# Autodesk Inventor assembly: robot
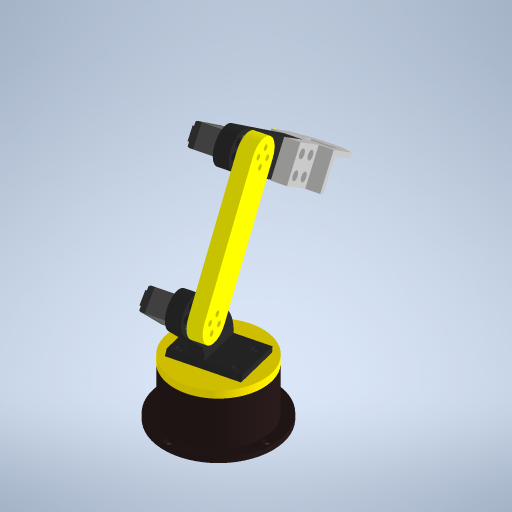
[picture p0: Inventor's stored thumbnail of the model, 512x512]
Saved by Autodesk Inventor 2024.2 (Build 282272000, 272)
## iProperties
Created: 2023-11-10
Part Number: robot
Document SubType Name: Assembly
Designer: nosal
Author: nosal
## Documents named in this file (8)
- C:\Users\nosal\OneDrive\Pulpit\projekty 3d\Inżynierka\Robot2\robot.iam
- C:\Users\nosal\OneDrive\Pulpit\projekty 3d\Inżynierka\Robot2\Podstawa1.ipt
- C:\Users\nosal\OneDrive\Pulpit\projekty 3d\Inżynierka\Robot2\silnik\MG_996R.iam
- C:\Users\nosal\OneDrive\Pulpit\projekty 3d\Inżynierka\Robot2\Podstawa2.ipt
- C:\Users\nosal\OneDrive\Pulpit\projekty 3d\Inżynierka\Robot2\Ramie1.ipt
- C:\Users\nosal\OneDrive\Pulpit\projekty 3d\Inżynierka\Robot2\Ramie2.ipt
- C:\Users\nosal\OneDrive\Pulpit\projekty 3d\Inżynierka\Robot2\Ramie3.ipt
- C:\Users\nosal\OneDrive\Pulpit\projekty 3d\Inżynierka\Robot2\chwytak\podstawachwytak.ipt
## Components (9 placed, 7 different names)
1. Podstawa1:1 — Sztywne:1
2. MG_996R:1 [sub-assembly] — Sztywne:1, Obrotowe:1
3. Podstawa2:1 — Obrotowe:1, Sztywne:2
4. Ramie1:1 — Sztywne:2, Obrotowe:2, Sztywne:3
5. MG_996R:2 [sub-assembly] — Obrotowe:2, Sztywne:3, Obrotowe:3
6. Ramie2:1 — Obrotowe:3, Obrotowe:4
7. Ramie3:1 — Sztywne:4, Sztywne:5
8. MG_996R:3 [sub-assembly] — Sztywne:4, Obrotowe:4
9. podstawachwytak:1 — Sztywne:5
## Relationships (9: WeldJoint 5, RevoluteJoint 4)
- Sztywne:1 [WeldJoint]: Podstawa1:1 ↔ MG_996R:1
- Obrotowe:1 [RevoluteJoint]: MG_996R:1 ↔ Podstawa2:1
- Sztywne:2 [WeldJoint]: Podstawa2:1 ↔ Ramie1:1
- Obrotowe:2 [RevoluteJoint]: Ramie1:1 ↔ MG_996R:2
- Sztywne:3 [WeldJoint]: Ramie1:1 ↔ MG_996R:2
- Obrotowe:3 [RevoluteJoint]: MG_996R:2 ↔ Ramie2:1
- Sztywne:4 [WeldJoint]: Ramie3:1 ↔ MG_996R:3
- Obrotowe:4 [RevoluteJoint]: Ramie2:1 ↔ MG_996R:3
- Sztywne:5 [WeldJoint]: Ramie3:1 ↔ podstawachwytak:1
